# Autodesk Inventor assembly: ＠ArmHD2019
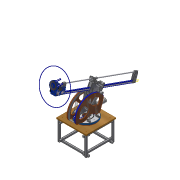
[picture p0: Inventor's stored thumbnail of the model, 180x180]
Saved by Autodesk Inventor 2019.4 (Build 234330000, 330)
## iProperties
Created: 2018-08-09
Part Number: ＠ArmHD2019
Document SubType Name: Assembly
Designer: Owner
Mass: 3480.12 g
Surface Area: 17809.2 cm^2
Volume: 3279.54 cm^3
Density: 1.06116 g/cm^3
Author: Owner
## Documents named in this file (33)
- E:\ロボ研\キャチロボ\キャチロボ2019\アーム2019\2019HDarm\＠ArmHD2019.iam
- E:\ロボ研\キャチロボ\キャチロボ2019\アーム2019\2019HDarm\Slide_1.iam
- E:\ロボ研\キャチロボ\キャチロボ2019\アーム2019\2019HDarm\Robot_Base.iam
- E:\ロボ研\キャチロボ\キャチロボ2019\アーム2019\2019HDarm\Joint_1.iam
- E:\ロボ研\キャチロボ\キャチロボ2018\アーム\アーム01\回路ボックス.iam
- E:\ロボ研\キャチロボ\キャチロボ2019\アーム2019\2019HDarm\Joint_3.iam
- E:\ロボ研\キャチロボ\キャチロボ2019\アーム2019\2019HDarm\Pitch_B.ipt
- E:\ロボ研\キャチロボ\キャチロボ2019\アーム2019\2019HDarm\p8-19flange.ipt
- E:\ロボ研\キャチロボ\キャチロボ2019\アーム2019\2019HDarm\p8ALshaft.ipt
- E:\ロボ研\キャチロボ\キャチロボ2019\アーム2019\KHK_SUMA120SUMA120On\AIS2019\SUMA1-20_SUMA1-20_On.iam
- E:\ロボ研\キャチロボ\キャチロボ2019\アーム2019\2019HDarm\RS555PH_Geared_Motor.ipt
- E:\ロボ研\キャチロボ\キャチロボ2019\アーム2019\PitchGears\PitchGears.iam
- E:\ロボ研\キャチロボ\キャチロボ2019\アーム2019\PitchGears\PitchSquarePipe.ipt
- E:\ロボ研\キャチロボ\キャチロボ2019\アーム2019\PitchGears\PitchSquarePipe2.ipt
- E:\ロボ研\キャチロボ\キャチロボ2019\アーム2019\PitchGears\RailWay.ipt
- E:\ロボ研\キャチロボ\キャチロボ2019\アーム2019\SqPipeminin.ipt
- E:\ロボ研\キャチロボ\キャチロボ2019\アーム2019\SqPipe92.ipt
- E:\ロボ研\キャチロボ\キャチロボ2019\アーム2019\Tplate.ipt
- E:\ロボ研\キャチロボ\キャチロボ2019\アーム2019\支え.ipt
- E:\ロボ研\キャチロボ\キャチロボ2019\アーム2019\p9ALshaft.ipt
- E:\ロボ研\キャチロボ\キャチロボ2019\アーム2019\Tplate_L.ipt
- E:\ロボ研\キャチロボ\キャチロボ2019\アーム2019\p8-10_OilessFlange.ipt
- E:\ロボ研\キャチロボ\キャチロボ2019\アーム2019\p8l65ALshaft.ipt
- E:\ロボ研\キャチロボ\キャチロボ2019\アーム2019\RS555-71K_MotorsupportAL.ipt
- E:\ロボ研\キャチロボ\キャチロボ2019\アーム2019\RS555-71K_MotorsupportPolica.ipt
- E:\ロボ研\キャチロボ\キャチロボ2019\アーム2019\2019HDarm\p8ALshaftP.ipt
- E:\ロボ研\キャチロボ\キャチロボ2019\アーム2019\2019HDarm\Key1.ipt
- E:\ロボ研\キャチロボ\キャチロボ2018\アーム\ポテンショメータB.ipt
- E:\ロボ研\キャチロボ\キャチロボ2018\アーム\アーム01\2axsisSensGear.ipt
- E:\ロボ研\キャチロボ\キャチロボ2019\アーム2019\2019HDarm\FleLG.ipt
- E:\ロボ研\キャチロボ\キャチロボ2019\Slide_2_ver2.iam
- E:\ロボ研\キャチロボ\キャチロボ2019\Joint_2_ver2.iam
- E:\ロボ研\キャチロボ\キャチロボ2019\手首関節.iam
## Components (51 placed, 32 different names)
1. Slide_1:1 [sub-assembly] — 設計用拘束, スライダ:3, 設計用, 設計用3, リジッド:15
2. Robot_Base:1 [sub-assembly] — フラッシュ:3, 挿入:1, 挿入:2, 設計用, 回転:11
3. Joint_1:1 [sub-assembly] — Fit, 挿入:16, 挿入:17, 角度:3, 挿入:22, 挿入:23, 挿入:43, 回転:3, 回転:11
4. 回路ボックス:1 [sub-assembly] — 挿入:1, 挿入:2
5. Joint_3:1 [sub-assembly] — スライダ:3, 設計用2, メイト:7, メイト:8, メイト:19, メイト:23, 正接:1, 挿入:36, 挿入:37, 挿入:38, 挿入:39, 回転:10
6. Pitch_B:1 — 設計用2, メイト:15, フラッシュ:7, メイト:16, 挿入:16, 挿入:17, 挿入:25, 挿入:26, 挿入:27, メイト:26, リジッド:6, リジッド:7, 挿入:47
7. p8ALshaft:1 — メイト:7, メイト:8, メイト:10, メイト:25, メイト:26, フラッシュ:11, メイト:27
8. SUMA1-20_SUMA1-20_On:1 [sub-assembly] — 挿入:3, メイト:15
9. RS555PH_Geared_Motor:1 — 挿入:3, フラッシュ:7, フラッシュ:10, リジッド:5
10. PitchGears:1 [sub-assembly] — メイト:10, Fit, メイト:16, 挿入:18, 挿入:19, 挿入:20, 挿入:21, 挿入:35, 挿入:49, 挿入:50
11. PitchGears:2 [sub-assembly] — 挿入:40, 挿入:42, メイト:28, 回転:5, 回転:6
12. PitchSquarePipe2:1 — 挿入:18, 挿入:19
13. PitchSquarePipe:1 — 挿入:20, 挿入:21, メイト:19, メイト:23
14. RailWay:1 — 角度:3, 正接:1, メイト:25, 挿入:44
15. Tplate:1 — リジッド:1, リジッド:10, フラッシュ:11
16. 支え:1 — 挿入:25, 挿入:26, 挿入:27, 挿入:28, 挿入:29, 挿入:30, リジッド:1, 挿入:46
17. p9ALshaft:1 — 挿入:28
18. p9ALshaft:2 — 挿入:29
19. p9ALshaft:3 — 挿入:30
20. Tplate_L:1 — 挿入:33, 挿入:34, リジッド:11, 挿入:48, 回転:2, 回転:4, 回転:8, 回転:9
21. RailWay:2 — 挿入:33, 挿入:34, 挿入:45
22. p8-10_OilessFlange:1 — 挿入:41
23. p8-10_OilessFlange:2 — 挿入:51
24. p8-19flange:1 — 挿入:35
25. PitchSquarePipe2:2 — 挿入:38, 挿入:39
26. PitchSquarePipe:2 — 挿入:36, 挿入:37, 挿入:42
27. p8-19flange:3 — 挿入:40, 挿入:41, メイト:27
28. Pitch_B:2 — 挿入:43, 回転:2, 回転:3, 回転:4, 挿入:51
29. p8l65ALshaft:1 — 挿入:44
30. p8l65ALshaft:2 — 挿入:45
31. SqPipe92:1 — リジッド:2
32. SqPipe92:2 — リジッド:3
33. RS555-71K_MotorsupportAL:1 — フラッシュ:10, リジッド:5, リジッド:6
34. RS555-71K_MotorsupportPolica:1 — リジッド:7
35. SqPipe92:3 — リジッド:10
36. SqPipe92:4 — リジッド:11
37. p8-10_OilessFlange:3 — 挿入:46
38. p8-10_OilessFlange:4 — 挿入:47
39. p8ALshaftP:1 — 挿入:48, フラッシュ:12, メイト:28, リジッド:12
40. Key1:1 — フラッシュ:12, 挿入:49, 挿入:50
41. Key1:2 — リジッド:12, 回転:5, 回転:6
42. 2axsisSensGear:1 — 正接:2
43. ポテンショメータB:2 — 回転:10
44. FleLG:1 — 回転:8, 回転:9, 正接:2
45. Slide_2_ver2:3 [sub-assembly] — リジッド:13, リジッド:14
46. Joint_2_ver2:2 [sub-assembly] — リジッド:14
47. 手首関節:1 [sub-assembly] — リジッド:13, リジッド:15
48. SqPipeminin:2 — 挿入:22, 挿入:23
49. SqPipeminin:3
50. SqPipeminin:4 — リジッド:2
51. SqPipeminin:5 — リジッド:3
## Component patterns: (4 elements, first: SqPipeminin:2)
## Relationships (85: Insert 36, Mate 13, WeldJoint 12, RevoluteJoint 10, Flush 9, Angle 2, Tangent 2, TranslationJoint 1)
- [Flush]: Robot_Base:1
- [Flush]: Robot_Base:1
- フラッシュ:3 [Flush]: Robot_Base:1
- 挿入:1 [Insert]: Robot_Base:1 ↔ 回路ボックス:1
- 挿入:2 [Insert]: Robot_Base:1 ↔ 回路ボックス:1
- スライダ:3 [TranslationJoint]: Slide_1:1 ↔ Joint_3:1
- 設計用拘束 [Mate]: Slide_1:1
- 設計用 [Mate] (40 mm): Slide_1:1 ↔ Robot_Base:1
- 設計用3 [Flush]: Slide_1:1
- 設計用2 [Flush]: Joint_3:1 ↔ Pitch_B:1
- メイト:7 [Mate] (134 mm): Joint_3:1 ↔ p8ALshaft:1
- メイト:8 [Mate] (134 mm): Joint_3:1 ↔ p8ALshaft:1
- 挿入:3 [Insert] (-2 mm): SUMA1-20_SUMA1-20_On:1 ↔ RS555PH_Geared_Motor:1
- メイト:10 [Mate]: p8ALshaft:1 ↔ PitchGears:1
- Fit [Angle] (0 deg): Joint_1:1 ↔ PitchGears:1
- メイト:15 [Mate]: Pitch_B:1 ↔ SUMA1-20_SUMA1-20_On:1
- フラッシュ:7 [Flush]: Pitch_B:1 ↔ RS555PH_Geared_Motor:1
- メイト:16 [Mate]: Pitch_B:1 ↔ PitchGears:1
- 挿入:16 [Insert]: Joint_1:1 ↔ Pitch_B:1
- 挿入:17 [Insert]: Joint_1:1 ↔ Pitch_B:1
- 挿入:18 [Insert]: PitchGears:1 ↔ PitchSquarePipe2:1
- 挿入:19 [Insert]: PitchGears:1 ↔ PitchSquarePipe2:1
- 挿入:20 [Insert]: PitchGears:1 ↔ PitchSquarePipe:1
- 挿入:21 [Insert]: PitchGears:1 ↔ PitchSquarePipe:1
- メイト:19 [Mate]: Joint_3:1 ↔ PitchSquarePipe:1
- メイト:23 [Mate]: Joint_3:1 ↔ PitchSquarePipe:1
- 角度:3 [Angle] (90 deg): Joint_1:1 ↔ RailWay:1
- 正接:1 [Tangent]: Joint_3:1 ↔ RailWay:1
- メイト:25 [Mate]: p8ALshaft:1 ↔ RailWay:1
- 挿入:22 [Insert]: Joint_1:1 ↔ SqPipeminin:2
- 挿入:23 [Insert]: Joint_1:1 ↔ SqPipeminin:2
- 挿入:25 [Insert] (20 mm): Pitch_B:1 ↔ 支え:1
- 挿入:26 [Insert] (20 mm): Pitch_B:1 ↔ 支え:1
- 挿入:27 [Insert] (20 mm): Pitch_B:1 ↔ 支え:1
- 挿入:28 [Insert]: 支え:1 ↔ p9ALshaft:1
- 挿入:29 [Insert]: 支え:1 ↔ p9ALshaft:2
- 挿入:30 [Insert]: 支え:1 ↔ p9ALshaft:3
- リジッド:1 [WeldJoint]: Tplate:1 ↔ 支え:1
- 挿入:33 [Insert]: Tplate_L:1 ↔ RailWay:2
- 挿入:34 [Insert]: Tplate_L:1 ↔ RailWay:2
- 挿入:35 [Insert]: PitchGears:1 ↔ p8-19flange:1
- 挿入:36 [Insert]: Joint_3:1 ↔ PitchSquarePipe:2
- 挿入:37 [Insert]: Joint_3:1 ↔ PitchSquarePipe:2
- 挿入:38 [Insert]: Joint_3:1 ↔ PitchSquarePipe2:2
- 挿入:39 [Insert]: Joint_3:1 ↔ PitchSquarePipe2:2
- 挿入:40 [Insert]: PitchGears:2 ↔ p8-19flange:3
- メイト:26 [Mate]: Pitch_B:1 ↔ p8ALshaft:1
- 挿入:41 [Insert] (-0.5 mm): p8-10_OilessFlange:1 ↔ p8-19flange:3
- 挿入:42 [Insert]: PitchGears:2 ↔ PitchSquarePipe:2
- 挿入:43 [Insert]: Joint_1:1 ↔ Pitch_B:2
- 挿入:44 [Insert]: RailWay:1 ↔ p8l65ALshaft:1
- 挿入:45 [Insert]: RailWay:2 ↔ p8l65ALshaft:2
- リジッド:2 [WeldJoint]: SqPipe92:1 ↔ SqPipeminin:4
- リジッド:3 [WeldJoint]: SqPipe92:2 ↔ SqPipeminin:5
- フラッシュ:10 [Flush]: RS555PH_Geared_Motor:1 ↔ RS555-71K_MotorsupportAL:1
- リジッド:5 [WeldJoint]: RS555PH_Geared_Motor:1 ↔ RS555-71K_MotorsupportAL:1
- リジッド:6 [WeldJoint]: Pitch_B:1 ↔ RS555-71K_MotorsupportAL:1
- リジッド:7 [WeldJoint]: Pitch_B:1 ↔ RS555-71K_MotorsupportPolica:1
- リジッド:10 [WeldJoint]: Tplate:1 ↔ SqPipe92:3
- リジッド:11 [WeldJoint]: Tplate_L:1 ↔ SqPipe92:4
- 挿入:46 [Insert]: 支え:1 ↔ p8-10_OilessFlange:3
- 挿入:47 [Insert]: Pitch_B:1 ↔ p8-10_OilessFlange:4
- フラッシュ:11 [Flush]: p8ALshaft:1 ↔ Tplate:1
- 挿入:48 [Insert]: Tplate_L:1 ↔ p8ALshaftP:1
- フラッシュ:12 [Flush]: p8ALshaftP:1 ↔ Key1:1
- 挿入:49 [Insert]: PitchGears:1 ↔ Key1:1
- 挿入:50 [Insert]: PitchGears:1 ↔ Key1:1
- 回転:2 [RevoluteJoint]: Tplate_L:1 ↔ Pitch_B:2
- 回転:3 [RevoluteJoint]: Joint_1:1 ↔ Pitch_B:2
- 回転:4 [RevoluteJoint]: Tplate_L:1 ↔ Pitch_B:2
- メイト:27 [Mate]: p8ALshaft:1 ↔ p8-19flange:3
- メイト:28 [Mate]: PitchGears:2 ↔ p8ALshaftP:1
- リジッド:12 [WeldJoint]: p8ALshaftP:1 ↔ Key1:2
- 回転:5 [RevoluteJoint]: PitchGears:2 ↔ Key1:2
- 回転:6 [RevoluteJoint]: PitchGears:2 ↔ Key1:2
- [RevoluteJoint] (-1 mm): 2axsisSensGear:1 ↔ ポテンショメータB:2
- 回転:8 [RevoluteJoint]: Tplate_L:1 ↔ FleLG:1
- 回転:9 [RevoluteJoint]: Tplate_L:1 ↔ FleLG:1
- 正接:2 [Tangent]: 2axsisSensGear:1 ↔ FleLG:1
- 回転:10 [RevoluteJoint]: Joint_3:1 ↔ ポテンショメータB:2
- 挿入:51 [Insert]: p8-10_OilessFlange:2 ↔ Pitch_B:2
- 回転:11 [RevoluteJoint]: Robot_Base:1 ↔ Joint_1:1
- リジッド:13 [WeldJoint]: Slide_2_ver2:3 ↔ 手首関節:1
- リジッド:14 [WeldJoint]: Slide_2_ver2:3 ↔ Joint_2_ver2:2
- リジッド:15 [WeldJoint]: Slide_1:1 ↔ 手首関節:1
